# Autodesk Inventor assembly: Assembly6
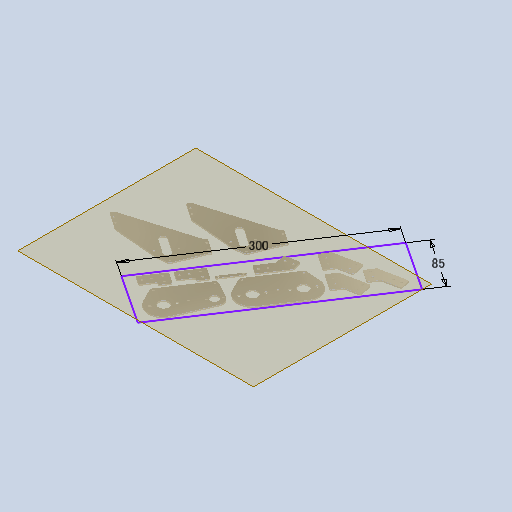
[picture p0: Inventor's stored thumbnail of the model, 512x512]
Saved by Autodesk Inventor 2025.2 (Build 292293000, 293)
## iProperties
Created: 2024-12-19
Part Number: Assembly6
Document SubType Name: Assembly
Designer: haruy
Author: haruy
## Documents named in this file (8)
- C:\Users\haruy\Documents\ロボコン\NHK2025\cad\cnc\Assembly6.iam
- C:\Users\haruy\Documents\ロボコン\NHK2025\cad\nagahisa\belt_liner\belt_liner_v1_Plate_4.ipt
- C:\Users\haruy\Documents\ロボコン\NHK2025\cad\nagahisa\belt_liner\belt_liner_v1_Plate_5.ipt
- C:\Users\haruy\Documents\ロボコン\NHK2025\cad\nagahisa\belt_liner\belt_liner_v1_Plate_14.ipt
- C:\Users\haruy\Documents\ロボコン\NHK2025\cad\nagahisa\belt_liner\belt_liner_v1_Plate_8.ipt
- C:\Users\haruy\Documents\ロボコン\NHK2025\cad\nagahisa\belt_liner\belt_liner_v1_Plate_13.ipt
- C:\Users\haruy\Documents\ロボコン\NHK2025\cad\nagahisa\belt_liner\belt_liner_v1_Plate_12.ipt
- C:\Users\haruy\Documents\ロボコン\NHK2025\cad\nagahisa\belt_liner\belt_liner_v1_Plate_11.ipt
## Components (11 placed, 7 different names)
1. belt_liner_v1_Plate_4:1 — フラッシュ:1, フラッシュ:12, メイト:4
2. belt_liner_v1_Plate_5:1 — フラッシュ:2, フラッシュ:12, メイト:1, メイト:2
3. belt_liner_v1_Plate_14:1 — フラッシュ:3, フラッシュ:15
4. belt_liner_v1_Plate_8:1 — フラッシュ:4, フラッシュ:13
5. belt_liner_v1_Plate_8:2 — フラッシュ:5, メイト:1, フラッシュ:13
6. belt_liner_v1_Plate_13:1 — フラッシュ:6
7. belt_liner_v1_Plate_13:2 — フラッシュ:7, メイト:4
8. belt_liner_v1_Plate_12:1 — フラッシュ:9, メイト:2, フラッシュ:14, メイト:3
9. belt_liner_v1_Plate_12:2 — フラッシュ:8, フラッシュ:14, メイト:3, フラッシュ:15
10. belt_liner_v1_Plate_11:1 — フラッシュ:10, フラッシュ:16
11. belt_liner_v1_Plate_11:2 — フラッシュ:11, フラッシュ:16
## Relationships (20: Flush 16, Mate 4)
- フラッシュ:1 [Flush]: belt_liner_v1_Plate_4:1
- フラッシュ:2 [Flush]: belt_liner_v1_Plate_5:1
- フラッシュ:3 [Flush]: belt_liner_v1_Plate_14:1
- フラッシュ:4 [Flush]: belt_liner_v1_Plate_8:1
- フラッシュ:5 [Flush]: belt_liner_v1_Plate_8:2
- フラッシュ:6 [Flush]: belt_liner_v1_Plate_13:1
- フラッシュ:7 [Flush]: belt_liner_v1_Plate_13:2
- フラッシュ:8 [Flush]: belt_liner_v1_Plate_12:2
- フラッシュ:9 [Flush]: belt_liner_v1_Plate_12:1
- フラッシュ:10 [Flush]: belt_liner_v1_Plate_11:1
- フラッシュ:11 [Flush]: belt_liner_v1_Plate_11:2
- フラッシュ:12 [Flush]: belt_liner_v1_Plate_4:1 ↔ belt_liner_v1_Plate_5:1
- メイト:1 [Mate] (50 mm): belt_liner_v1_Plate_5:1 ↔ belt_liner_v1_Plate_8:2
- フラッシュ:13 [Flush]: belt_liner_v1_Plate_8:1 ↔ belt_liner_v1_Plate_8:2
- メイト:2 [Mate] (5 mm): belt_liner_v1_Plate_5:1 ↔ belt_liner_v1_Plate_12:1
- フラッシュ:14 [Flush]: belt_liner_v1_Plate_12:1 ↔ belt_liner_v1_Plate_12:2
- メイト:3 [Mate] (5 mm): belt_liner_v1_Plate_12:1 ↔ belt_liner_v1_Plate_12:2
- フラッシュ:15 [Flush]: belt_liner_v1_Plate_14:1 ↔ belt_liner_v1_Plate_12:2
- メイト:4 [Mate] (5 mm): belt_liner_v1_Plate_4:1 ↔ belt_liner_v1_Plate_13:2
- フラッシュ:16 [Flush]: belt_liner_v1_Plate_11:1 ↔ belt_liner_v1_Plate_11:2
